# Autodesk Inventor assembly: CameraMountedOnBot
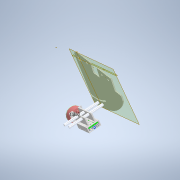
[picture p0: Inventor's stored thumbnail of the model, 180x180]
Saved by Autodesk Inventor 2020 (Build 240168000, 168)
## iProperties
Created: 2020-02-08
Part Number: CameraMountedOnBot
Document SubType Name: Assembly
Designer: Chris Gerth
Author: Chris Gerth
## Documents named in this file (12)
- C:\Users\Chris Gerth\Documents\Robotics\RobotCasserole2020\piVisionCase\CameraMountedOnBot.iam
- C:\Users\Chris Gerth\Documents\Robotics\RobotCasserole2020\piVisionCase\ypieceforconnectingbracehood.ipt
- C:\Users\Chris Gerth\Documents\Robotics\RobotCasserole2020\piVisionCase\8-5churro.ipt
- C:\Users\Chris Gerth\Documents\Robotics\RobotCasserole2020\piVisionCase\cameraToChurroSplineRight.ipt
- C:\Users\Chris Gerth\Documents\Robotics\RobotCasserole2020\piVisionCase\cameraToChurroSplineLeft.ipt
- C:\Users\Chris Gerth\Documents\Robotics\RobotCasserole2020\piVisionCase\camHolderTop.ipt
- C:\Users\Chris Gerth\Documents\Robotics\RobotCasserole2020\piVisionCase\camHolderBottom.ipt
- C:\Users\Chris Gerth\Documents\Robotics\RobotCasserole2020\piVisionCase\camera.ipt
- C:\Users\Chris Gerth\Documents\Robotics\RobotCasserole2020\piVisionCase\ledRing.ipt
- C:\Users\Chris Gerth\Documents\Robotics\RobotCasserole2020\piVisionCase\piBottom.ipt
- C:\Users\Chris Gerth\Documents\Robotics\RobotCasserole2020\piVisionCase\Raspberry Pi 4 Model B.iam
- C:\Users\Chris Gerth\Documents\Robotics\RobotCasserole2020\piVisionCase\piTop.ipt
## Components (12 placed, 11 different names)
1. ypieceforconnectingbracehood:1 — Mate:1, Mate:2, Flush:1, Flush:2, Mate:3, Mate:4
2. 8-5churro:1 — Mate:1, Mate:2, Flush:1, Mate:5, Mate:8
3. 8-5churro:2 — Flush:2, Mate:3, Mate:4, Mate:6, Mate:7
4. cameraToChurroSplineRight:1 — Mate:7, Mate:8, Mate:19, Mate:22, Mate:24
5. cameraToChurroSplineLeft:1 — Mate:5, Mate:6, Mate:11, Mate:23, Mate:25
6. camHolderTop:1 — Mate:17, Mate:18, Mate:19, Mate:20
7. camHolderBottom:1 — Mate:11, Mate:14, Mate:15, Mate:16, Mate:17, Mate:18, Mate:22
8. camera:1 — Mate:14, Mate:15, Mate:16, Mate:21
9. ledRing:1 — Mate:20, Mate:21
10. piBottom:1 — Mate:23, Mate:24, Mate:25, Mate:26, Mate:27, Mate:28, Mate:29, Flush:3, Flush:4
11. Raspberry Pi 4 Model B:1 [sub-assembly] — Mate:26, Mate:27, Mate:28
12. piTop:1 — Mate:29, Flush:3, Flush:4
## Relationships (29: Mate 25, Flush 4)
- Mate:1: ypieceforconnectingbracehood:1 ↔ 8-5churro:1
- Mate:2: ypieceforconnectingbracehood:1 ↔ 8-5churro:1
- Flush:1: ypieceforconnectingbracehood:1 ↔ 8-5churro:1
- Flush:2: ypieceforconnectingbracehood:1 ↔ 8-5churro:2
- Mate:3: ypieceforconnectingbracehood:1 ↔ 8-5churro:2
- Mate:4: ypieceforconnectingbracehood:1 ↔ 8-5churro:2
- Mate:5: 8-5churro:1 ↔ cameraToChurroSplineLeft:1
- Mate:6: 8-5churro:2 ↔ cameraToChurroSplineLeft:1
- Mate:7: 8-5churro:2 ↔ cameraToChurroSplineRight:1
- Mate:8: 8-5churro:1 ↔ cameraToChurroSplineRight:1
- Mate:11: cameraToChurroSplineLeft:1 ↔ camHolderBottom:1
- Mate:14: camHolderBottom:1 ↔ camera:1
- Mate:15: camHolderBottom:1 ↔ camera:1
- Mate:16: camHolderBottom:1 ↔ camera:1
- Mate:17: camHolderTop:1 ↔ camHolderBottom:1
- Mate:18: camHolderTop:1 ↔ camHolderBottom:1
- Mate:19: cameraToChurroSplineRight:1 ↔ camHolderTop:1
- Mate:20: camHolderTop:1 ↔ ledRing:1
- Mate:21: camera:1 ↔ ledRing:1
- Mate:22: cameraToChurroSplineRight:1 ↔ camHolderBottom:1
- Mate:23: cameraToChurroSplineLeft:1 ↔ piBottom:1
- Mate:24: cameraToChurroSplineRight:1 ↔ piBottom:1
- Mate:25: cameraToChurroSplineLeft:1 ↔ piBottom:1
- Mate:26: piBottom:1 ↔ Raspberry Pi 4 Model B:1
- Mate:27 (6.35 mm): piBottom:1 ↔ Raspberry Pi 4 Model B:1
- Mate:28: piBottom:1 ↔ Raspberry Pi 4 Model B:1
- Mate:29: piBottom:1 ↔ piTop:1
- Flush:3: piBottom:1 ↔ piTop:1
- Flush:4: piBottom:1 ↔ piTop:1
